# Autodesk Inventor assembly: tale connection
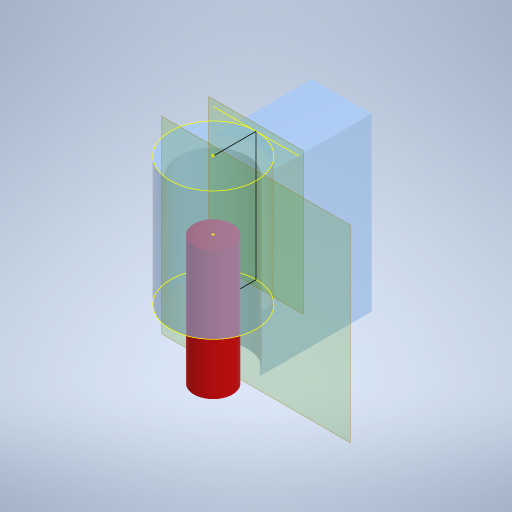
[picture p0: Inventor's stored thumbnail of the model, 512x512]
Saved by Autodesk Inventor 2023 (Build 270158000, 158)
## iProperties
Created: 2022-10-23
Part Number: tale connection
Document SubType Name: Assembly
Designer: ellie
Author: ellie
## Documents named in this file (3)
- C:\Users\ellie\Documents\github\tanekonsat2022_runback\machinary\body\tale connection.iam
- C:\Users\ellie\Documents\github\tanekonsat2022_runback\machinary\body\tale inner.ipt
- C:\Users\ellie\Documents\github\tanekonsat2022_runback\machinary\body\tale outer.ipt
## Components (2 placed, 2 different names)
1. tale inner:1 — メイト:1, メイト:2
2. tale outer:1 — メイト:1, メイト:2, フラッシュ:1
## Relationships (3: Mate 2, Flush 1)
- メイト:1 [Mate] (6 mm): tale inner:1 ↔ tale outer:1
- メイト:2 [Mate]: tale inner:1 ↔ tale outer:1
- フラッシュ:1 [Flush]: tale outer:1
